# Autodesk Inventor assembly: cardSpool
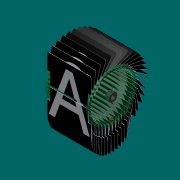
[picture p0: Inventor's stored thumbnail of the model, 180x180]
Saved by Autodesk Inventor 2016 (Build 200138000, 138)
## iProperties
Created: 2015-10-05
Part Number: cardSpool
Document SubType Name: Assembly
Designer: Sawaiz
Author: Sawaiz
## Documents named in this file (47)
- C:\Users\sawaiz\oneDrive\projects\splitFlapDisplay\spool\cardSpool.iam
- C:\Users\sawaiz\oneDrive\projects\splitFlapDisplay\spool\spoolBase.ipt
- C:\Users\sawaiz\oneDrive\projects\splitFlapDisplay\cards\card-01.ipt
- C:\Users\sawaiz\oneDrive\projects\splitFlapDisplay\cards\card-02.ipt
- C:\Users\sawaiz\oneDrive\projects\splitFlapDisplay\cards\card-03.ipt
- C:\Users\sawaiz\oneDrive\projects\splitFlapDisplay\cards\card-04.ipt
- C:\Users\sawaiz\oneDrive\projects\splitFlapDisplay\cards\card-05.ipt
- C:\Users\sawaiz\oneDrive\projects\splitFlapDisplay\cards\card-06.ipt
- C:\Users\sawaiz\oneDrive\projects\splitFlapDisplay\cards\card-07.ipt
- C:\Users\sawaiz\oneDrive\projects\splitFlapDisplay\cards\card-08.ipt
- C:\Users\sawaiz\oneDrive\projects\splitFlapDisplay\cards\card-09.ipt
- C:\Users\sawaiz\oneDrive\projects\splitFlapDisplay\cards\card-10.ipt
- C:\Users\sawaiz\oneDrive\projects\splitFlapDisplay\cards\card-11.ipt
- C:\Users\sawaiz\oneDrive\projects\splitFlapDisplay\cards\card-12.ipt
- C:\Users\sawaiz\oneDrive\projects\splitFlapDisplay\cards\card-13.ipt
- C:\Users\sawaiz\oneDrive\projects\splitFlapDisplay\cards\card-14.ipt
- C:\Users\sawaiz\oneDrive\projects\splitFlapDisplay\cards\card-15.ipt
- C:\Users\sawaiz\oneDrive\projects\splitFlapDisplay\cards\card-16.ipt
- C:\Users\sawaiz\oneDrive\projects\splitFlapDisplay\cards\card-17.ipt
- C:\Users\sawaiz\oneDrive\projects\splitFlapDisplay\cards\card-18.ipt
- C:\Users\sawaiz\oneDrive\projects\splitFlapDisplay\cards\card-19.ipt
- C:\Users\sawaiz\oneDrive\projects\splitFlapDisplay\cards\card-20.ipt
- C:\Users\sawaiz\oneDrive\projects\splitFlapDisplay\cards\card-21.ipt
- C:\Users\sawaiz\oneDrive\projects\splitFlapDisplay\cards\card-22.ipt
- C:\Users\sawaiz\oneDrive\projects\splitFlapDisplay\cards\card-23.ipt
- C:\Users\sawaiz\oneDrive\projects\splitFlapDisplay\cards\card-24.ipt
- C:\Users\sawaiz\oneDrive\projects\splitFlapDisplay\cards\card-25.ipt
- C:\Users\sawaiz\oneDrive\projects\splitFlapDisplay\cards\card-26.ipt
- C:\Users\sawaiz\oneDrive\projects\splitFlapDisplay\cards\card-27.ipt
- C:\Users\sawaiz\oneDrive\projects\splitFlapDisplay\cards\card-28.ipt
- C:\Users\sawaiz\oneDrive\projects\splitFlapDisplay\cards\card-29.ipt
- C:\Users\sawaiz\oneDrive\projects\splitFlapDisplay\cards\card-30.ipt
- C:\Users\sawaiz\oneDrive\projects\splitFlapDisplay\cards\card-31.ipt
- C:\Users\sawaiz\oneDrive\projects\splitFlapDisplay\cards\card-32.ipt
- C:\Users\sawaiz\oneDrive\projects\splitFlapDisplay\cards\card-33.ipt
- C:\Users\sawaiz\oneDrive\projects\splitFlapDisplay\cards\card-34.ipt
- C:\Users\sawaiz\oneDrive\projects\splitFlapDisplay\cards\card-35.ipt
- C:\Users\sawaiz\oneDrive\projects\splitFlapDisplay\cards\card-36.ipt
- C:\Users\sawaiz\oneDrive\projects\splitFlapDisplay\cards\card-37.ipt
- C:\Users\sawaiz\oneDrive\projects\splitFlapDisplay\cards\card-38.ipt
- C:\Users\sawaiz\oneDrive\projects\splitFlapDisplay\cards\card-39.ipt
- C:\Users\sawaiz\oneDrive\projects\splitFlapDisplay\cards\card-40.ipt
- C:\Users\sawaiz\oneDrive\projects\splitFlapDisplay\spool\spoolGearSide.ipt
- C:\Users\sawaiz\oneDrive\projects\splitFlapDisplay\drive\gt236Tooth.ipt
- C:\Users\sawaiz\oneDrive\projects\splitFlapDisplay\drive\8mmShaftCollar.ipt
- C:\Users\sawaiz\oneDrive\projects\splitFlapDisplay\frame\magnet.ipt
- C:\Users\sawaiz\oneDrive\projects\splitFlapDisplay\parameters.xlsx
## Components (45 placed, 45 different names)
1. spoolBase:1 — Mate:4, Mate:5, Mate:6, Mate:7, Mate:8, Mate:9, Mate:10, Mate:11, Mate:12, Mate:13, Mate:14, Mate:15, Mate:16, Mate:17, Mate:18, Mate:19, Mate:20, Mate:21, Mate:22, Mate:23, Mate:24, Mate:25, Mate:26, Mate:27, Mate:28, Mate:29, Mate:30, Mate:31, Mate:32, Mate:33, Mate:34, Mate:35, Mate:36, Mate:37, Mate:38, Mate:39, Mate:40, Mate:41, Mate:42, Mate:43, Mate:44, Mate:45, Mate:46, Mate:50, Flush:40, Mate:51, Flush:41
2. spoolGearSide:1 — Mate:45, Mate:46, Mate:47, Mate:48, Mate:49
3. card-01:1 — Mate:4, Flush:1, Mate:44, Mate:47
4. card-02:1 — Mate:5, Flush:1, Flush:2
5. card-03:1 — Mate:6, Flush:2, Flush:3
6. card-04:1 — Mate:7, Flush:3, Flush:4
7. card-05:1 — Mate:8, Flush:4, Flush:5
8. card-06:1 — Mate:9, Flush:5, Flush:6
9. card-07:1 — Mate:10, Flush:6, Flush:7
10. card-08:1 — Mate:11, Flush:7, Flush:8
11. card-09:1 — Mate:12, Flush:8, Flush:9
12. card-10:1 — Mate:13, Flush:9, Flush:10
13. card-11:1 — Mate:14, Flush:10, Flush:11
14. card-12:1 — Mate:15, Flush:11, Flush:12
15. card-13:1 — Mate:16, Flush:12, Flush:13
16. card-14:1 — Mate:17, Flush:13, Flush:14
17. card-15:1 — Mate:18, Flush:14, Flush:15
18. card-16:1 — Mate:19, Flush:15, Flush:16
19. card-17:1 — Mate:20, Flush:16, Flush:17
20. card-18:1 — Mate:21, Flush:17, Flush:18
21. card-19:1 — Mate:22, Flush:18, Flush:19
22. card-20:1 — Mate:23, Flush:19, Flush:20, Flush:21
23. card-21:1 — Mate:24, Flush:20
24. card-22:1 — Mate:25, Flush:21, Flush:38
25. card-23:1 — Mate:26, Flush:37, Flush:38
26. card-24:1 — Mate:27, Flush:36, Flush:37
27. card-25:1 — Mate:28, Flush:35, Flush:36
28. card-26:1 — Mate:29, Flush:34, Flush:35
29. card-27:1 — Mate:30, Flush:33, Flush:34
30. card-28:1 — Mate:31, Flush:32, Flush:33
31. card-29:1 — Mate:32, Flush:31, Flush:32
32. card-30:1 — Mate:33, Flush:30, Flush:31
33. card-31:1 — Mate:34, Flush:29, Flush:30
34. card-32:1 — Mate:35, Flush:28, Flush:29
35. card-33:1 — Mate:36, Flush:27, Flush:28
36. card-34:1 — Mate:37, Flush:26, Flush:27
37. card-35:1 — Mate:38, Flush:25, Flush:26
38. card-36:1 — Mate:39, Flush:24, Flush:25
39. card-37:1 — Flush:39, Mate:43
40. card-38:1 — Flush:23, Flush:24, Mate:42, Flush:39
41. card-39:1 — Flush:22, Flush:23, Mate:41
42. card-40:1 — Flush:22, Mate:40
43. gt236Tooth:1 — Mate:48, Mate:49
44. 8mmShaftCollar:1 — Mate:50, Flush:40
45. magnet:1 — Mate:51, Flush:41
## Relationships (89: Mate 48, Flush 41)
- Mate:4: spoolBase:1 ↔ card-01:1
- Mate:5: spoolBase:1 ↔ card-02:1
- Mate:6: spoolBase:1 ↔ card-03:1
- Mate:7: spoolBase:1 ↔ card-04:1
- Mate:8: spoolBase:1 ↔ card-05:1
- Mate:9: spoolBase:1 ↔ card-06:1
- Mate:10: spoolBase:1 ↔ card-07:1
- Mate:11: spoolBase:1 ↔ card-08:1
- Mate:12: spoolBase:1 ↔ card-09:1
- Mate:13: spoolBase:1 ↔ card-10:1
- Mate:14: spoolBase:1 ↔ card-11:1
- Mate:15: spoolBase:1 ↔ card-12:1
- Mate:16: spoolBase:1 ↔ card-13:1
- Mate:17: spoolBase:1 ↔ card-14:1
- Mate:18: spoolBase:1 ↔ card-15:1
- Mate:19: spoolBase:1 ↔ card-16:1
- Mate:20: spoolBase:1 ↔ card-17:1
- Mate:21: spoolBase:1 ↔ card-18:1
- Mate:22: spoolBase:1 ↔ card-19:1
- Mate:23: spoolBase:1 ↔ card-20:1
- Mate:24: spoolBase:1 ↔ card-21:1
- Mate:25: spoolBase:1 ↔ card-22:1
- Flush:1: card-01:1 ↔ card-02:1
- Flush:2: card-02:1 ↔ card-03:1
- Flush:3: card-03:1 ↔ card-04:1
- Flush:4: card-04:1 ↔ card-05:1
- Flush:5: card-05:1 ↔ card-06:1
- Flush:6: card-06:1 ↔ card-07:1
- Flush:7: card-07:1 ↔ card-08:1
- Flush:8: card-08:1 ↔ card-09:1
- Flush:9: card-09:1 ↔ card-10:1
- Flush:10: card-10:1 ↔ card-11:1
- Flush:11: card-11:1 ↔ card-12:1
- Flush:12: card-12:1 ↔ card-13:1
- Flush:13: card-13:1 ↔ card-14:1
- Flush:14: card-14:1 ↔ card-15:1
- Flush:15: card-15:1 ↔ card-16:1
- Flush:16: card-16:1 ↔ card-17:1
- Flush:17: card-17:1 ↔ card-18:1
- Flush:18: card-18:1 ↔ card-19:1
- Flush:19: card-19:1 ↔ card-20:1
- Flush:20: card-20:1 ↔ card-21:1
- Flush:21: card-20:1 ↔ card-22:1
- Mate:26: spoolBase:1 ↔ card-23:1
- Mate:27: spoolBase:1 ↔ card-24:1
- Mate:28: spoolBase:1 ↔ card-25:1
- Mate:29: spoolBase:1 ↔ card-26:1
- Mate:30: spoolBase:1 ↔ card-27:1
- Mate:31: spoolBase:1 ↔ card-28:1
- Mate:32: spoolBase:1 ↔ card-29:1
- Mate:33: spoolBase:1 ↔ card-30:1
- Mate:34: spoolBase:1 ↔ card-31:1
- Mate:35: spoolBase:1 ↔ card-32:1
- Mate:36: spoolBase:1 ↔ card-33:1
- Mate:37: spoolBase:1 ↔ card-34:1
- Mate:38: spoolBase:1 ↔ card-35:1
- Mate:39: spoolBase:1 ↔ card-36:1
- Flush:22: card-39:1 ↔ card-40:1
- Flush:23: card-38:1 ↔ card-39:1
- Flush:24: card-36:1 ↔ card-38:1
- Flush:25: card-35:1 ↔ card-36:1
- Flush:26: card-34:1 ↔ card-35:1
- Flush:27: card-33:1 ↔ card-34:1
- Flush:28: card-32:1 ↔ card-33:1
- Flush:29: card-31:1 ↔ card-32:1
- Flush:30: card-30:1 ↔ card-31:1
- Flush:31: card-29:1 ↔ card-30:1
- Flush:32: card-28:1 ↔ card-29:1
- Flush:33: card-27:1 ↔ card-28:1
- Flush:34: card-26:1 ↔ card-27:1
- Flush:35: card-25:1 ↔ card-26:1
- Flush:36: card-24:1 ↔ card-25:1
- Flush:37: card-23:1 ↔ card-24:1
- Flush:38: card-22:1 ↔ card-23:1
- Mate:40: spoolBase:1 ↔ card-40:1
- Mate:41: spoolBase:1 ↔ card-39:1
- Mate:42: spoolBase:1 ↔ card-38:1
- Flush:39: card-37:1 ↔ card-38:1
- Mate:43: spoolBase:1 ↔ card-37:1
- Mate:44 (0.5 mm): spoolBase:1 ↔ card-01:1
- Mate:45: spoolBase:1 ↔ spoolGearSide:1
- Mate:46: spoolBase:1 ↔ spoolGearSide:1
- Mate:47 (0.5 mm): spoolGearSide:1 ↔ card-01:1
- Mate:48: spoolGearSide:1 ↔ gt236Tooth:1
- Mate:49: spoolGearSide:1 ↔ gt236Tooth:1
- Mate:50: spoolBase:1 ↔ 8mmShaftCollar:1
- Flush:40: spoolBase:1 ↔ 8mmShaftCollar:1
- Mate:51: spoolBase:1 ↔ magnet:1
- Flush:41: spoolBase:1 ↔ magnet:1
## Named parameters: height = 180 mm, width = 120 mm, depth = 120 mm, materialThickness = 3.175 mm, laserKerf = 0.12 mm, spoolDiameter = 90 mm, cardPinDiameter = 3 mm, cardNumber = 40, centeralShaftDiameter = 8 mm, cardWidth = 85.6 mm, cardHeight = 53.98 mm, cardThickness = 0.76 mm, cardFillet = 2.88 mm, cardCutoutHeight = 20 mm, cardSelected = 1, cardClearence = 0.5 mm, spoolHubDiameter = 20 mm, bearingOd = 22 mm, axleHegiht = 100 mm, bearingWidth = 8 mm, axleHeight = 95 mm, nutTrapwidth = 5.5 mm, nutTrapDepth = 2.5 mm, nutTrapClearence = 2 mm, beltLength = 240 mm, magnetLength = 3 mm, magnetDiameter = 6 mm, magnetProtusion = 0.25 mm, notchWidth = 10 mm, spoolThickness = 5.588 mm
